# Autodesk Inventor assembly: head_assembly
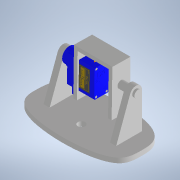
[picture p0: Inventor's stored thumbnail of the model, 180x180]
Saved by Autodesk Inventor 2020.3 (Build 243373000, 373)
## iProperties
Created: 2020-08-24
Part Number: head_assembly
Document SubType Name: Assembly
Designer: aditk
Author: aditk
## Documents named in this file (4)
- C:\Users\aditk\Desktop\PETcat\newCat\head_assembly.iam
- C:\Users\aditk\Desktop\PETcat\newCat\small_servo.iam
- C:\Users\aditk\Desktop\PETcat\newCat\head_mount.ipt
- C:\Users\aditk\Desktop\PETcat\newCat\head_p2.ipt
## Components (3 placed, 3 different names)
1. small_servo:1 [sub-assembly] — Mate:1, Mate:2, Mate:3, Insert:1
2. head_mount:1 — Insert:1
3. head_p2:1 — Mate:1, Mate:2, Mate:3
## Relationships (4: Mate 3, Insert 1)
- Mate:1: small_servo:1 ↔ head_p2:1
- Mate:2: small_servo:1 ↔ head_p2:1
- Mate:3: small_servo:1 ↔ head_p2:1
- Insert:1: small_servo:1 ↔ head_mount:1
